# Autodesk Inventor assembly: HF-Kabelführung-V3-XGantry
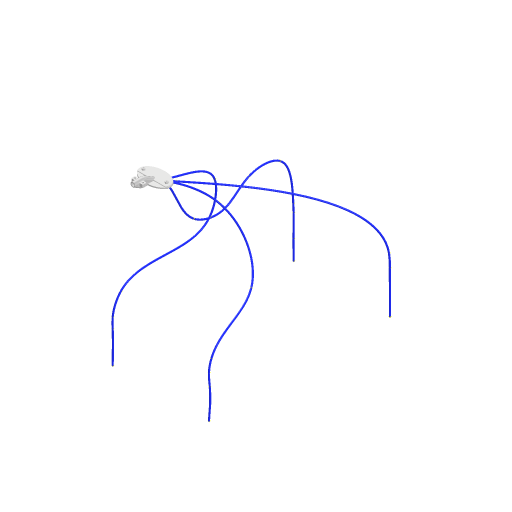
[picture p0: Inventor's stored thumbnail of the model, 512x512]
Saved by Autodesk Inventor 2023.2 (Build 272271000, 271)
## iProperties
Created: 2024-02-19
Part Number: HF-Kabelführung-V3-XGantry
Document SubType Name: Assembly
Designer: Nils Bade
Author: Nils Bade
## Documents named in this file (8)
- C:\Users\nilsb\Documents\Inventor\Projektarbeit-Bade\RatRig_Bade\HF-Kabelführung Measurement Chamber\HF-Kabelführung-V3-XGantry.iam
- C:\Users\nilsb\Documents\Inventor\Projektarbeit-Bade\RatRig_Bade\HF-Kabelführung Measurement Chamber\HF-Kabelführung-V3-XGantry-LängenSkizze.ipt
- C:\Users\nilsb\Documents\Inventor\Projektarbeit-Bade\RatRig_Bade\HF-Kabelführung Measurement Chamber\HF-Kabelführung-V3-XGantry\AIP\Kabel und Kabelbaum\HF-Kabelführung-V3-XGantry.Kabelbaum1.iam
- C:\Users\nilsb\Documents\Inventor\Projektarbeit-Bade\RatRig_Bade\HF-Kabelführung Measurement Chamber\HF-Kabelführung-V3-XGantry\AIP\Kabel und Kabelbaum\HF-Kabelführung-V3-XGantry.Kabelbaum-110.iam
- C:\Users\nilsb\Documents\Inventor\Projektarbeit-Bade\RatRig_Bade\HF-Kabelführung Measurement Chamber\HF-Kabeldurchführung-TopPanel-Base.ipt
- C:\Users\nilsb\Documents\Inventor\Projektarbeit-Bade\RatRig_Bade\HF-Kabelführung Measurement Chamber\HF-Kabeldurchführung-TopPanel-Deckel.ipt
- C:\Users\nilsb\Documents\Inventor\Projektarbeit-Bade\Schrauben\Cap Head Screw M4x12 - DIN912.ipt
- C:\Users\nilsb\Documents\Inventor\Projektarbeit-Bade\RatRig_Standards\Hex Nut - M4 DIN934.ipt
## Components (9 placed, 7 different names)
1. HF-Kabelführung-V3-XGantry-LängenSkizze:1 — Winkel:1, Passend:2, Passend:4
2. Kabelbaum - LILA 55 [sub-assembly]
3. HF-Kabelführung-V3-XGantry.Kabelbaum-110 [sub-assembly]
4. HF-Kabeldurchführung-TopPanel-Base:1 — Winkel:1, Passend:2, Passend:3, Fluchtend:1, Fluchtend:2, Passend:11, Passend:12
5. HF-Kabeldurchführung-TopPanel-Deckel:1 — Passend:3, Fluchtend:1, Fluchtend:2, Passend:4, Passend:5, Passend:6, Passend:7, Passend:8
6. Cap Head Screw M4x12 - DIN912:1 — Passend:5, Passend:8, Passend:9
7. Cap Head Screw M4x12 - DIN912:2 — Passend:6, Passend:7, Passend:10
8. Hex Nut - M4 DIN934:1 — Passend:9, Passend:12
9. Hex Nut - M4 DIN934:2 — Passend:10, Passend:11
## Relationships (14: Mate 11, Flush 2, Angle 1)
- Winkel:1 [Angle] (180 deg): HF-Kabelführung-V3-XGantry-LängenSkizze:1 ↔ HF-Kabeldurchführung-TopPanel-Base:1
- Passend:2 [Mate]: HF-Kabelführung-V3-XGantry-LängenSkizze:1 ↔ HF-Kabeldurchführung-TopPanel-Base:1
- Passend:3 [Mate]: HF-Kabeldurchführung-TopPanel-Base:1 ↔ HF-Kabeldurchführung-TopPanel-Deckel:1
- Fluchtend:1 [Flush]: HF-Kabeldurchführung-TopPanel-Base:1 ↔ HF-Kabeldurchführung-TopPanel-Deckel:1
- Fluchtend:2 [Flush]: HF-Kabeldurchführung-TopPanel-Base:1 ↔ HF-Kabeldurchführung-TopPanel-Deckel:1
- Passend:4 [Mate]: HF-Kabelführung-V3-XGantry-LängenSkizze:1 ↔ HF-Kabeldurchführung-TopPanel-Deckel:1
- Passend:5 [Mate]: HF-Kabeldurchführung-TopPanel-Deckel:1 ↔ Cap Head Screw M4x12 - DIN912:1
- Passend:6 [Mate]: HF-Kabeldurchführung-TopPanel-Deckel:1 ↔ Cap Head Screw M4x12 - DIN912:2
- Passend:7 [Mate]: HF-Kabeldurchführung-TopPanel-Deckel:1 ↔ Cap Head Screw M4x12 - DIN912:2
- Passend:8 [Mate]: HF-Kabeldurchführung-TopPanel-Deckel:1 ↔ Cap Head Screw M4x12 - DIN912:1
- Passend:9 [Mate]: Cap Head Screw M4x12 - DIN912:1 ↔ Hex Nut - M4 DIN934:1
- Passend:10 [Mate]: Cap Head Screw M4x12 - DIN912:2 ↔ Hex Nut - M4 DIN934:2
- Passend:11 [Mate] (3 mm): HF-Kabeldurchführung-TopPanel-Base:1 ↔ Hex Nut - M4 DIN934:2
- Passend:12 [Mate] (3 mm): HF-Kabeldurchführung-TopPanel-Base:1 ↔ Hex Nut - M4 DIN934:1
